# Autodesk Inventor assembly: Finger1
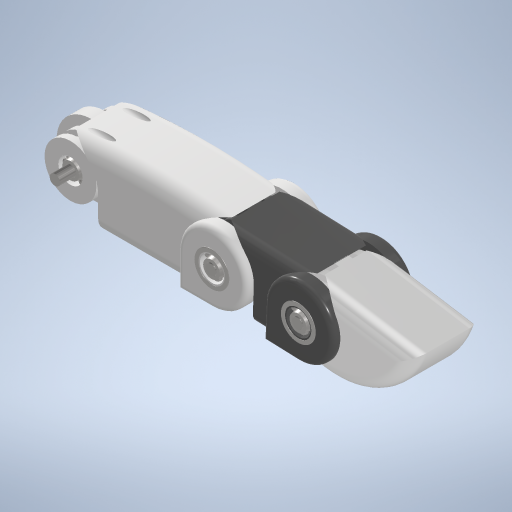
[picture p0: Inventor's stored thumbnail of the model, 512x512]
Saved by Autodesk Inventor 2024 (Build 280153000, 153)
## iProperties
Created: 2024-03-20
Part Number: Finger1
Document SubType Name: Assembly
Designer: Wojtek
Author: Wojtek
## Documents named in this file (6)
- D:\STUDIA\inventor Projects\Bionic_Hand\Fingers\Finger1.iam
- D:\STUDIA\inventor Projects\Bionic_Hand\Fingers\MiddlePart.ipt
- D:\STUDIA\inventor Projects\Bionic_Hand\Fingers\BottomPart.ipt
- C:\Users\Wojtek\OneDrive\Dokumenty\Inventor\Content Center Files\R2024\en-US\Bearing GB_T 292-2007\Rolling bearing B723 AC GB_T 292-2007.ipt
- D:\STUDIA\inventor Projects\Bionic_Hand\Fingers\Roller3mmx25mm.ipt
- D:\STUDIA\inventor Projects\Bionic_Hand\Fingers\TapPart.ipt
## Components (16 placed, 5 different names)
1. MiddlePart:1 — Rigid:1, Rigid:2, Rigid:3, Rigid:4
2. BottomPart:1 — Rigid:5, Rigid:6, Rigid:7, Rigid:8
3. Bearing GB/T 292-2007 Type IN - withdrawn B723 AC:1 — Rigid:1, Rotational:12
4. Bearing GB/T 292-2007 Type IN - withdrawn B723 AC:2 — Rigid:7
5. Bearing GB/T 292-2007 Type IN - withdrawn B723 AC:3 — Rigid:8, Rigid:10
6. Bearing GB/T 292-2007 Type IN - withdrawn B723 AC:4 — Rigid:2
7. Bearing GB/T 292-2007 Type IN - withdrawn B723 AC:5 — Rigid:4
8. Bearing GB/T 292-2007 Type IN - withdrawn B723 AC:6 — Rigid:5, Rigid:9
9. Bearing GB/T 292-2007 Type IN - withdrawn B723 AC:7 — Rigid:6
10. Bearing GB/T 292-2007 Type IN - withdrawn B723 AC:8 — Rigid:3, Rigid:12
11. Roller3mmx25mm:1 — Rigid:9, Rotational:12
12. Roller3mmx25mm:2 — Rigid:10
13. TapPart:1 — Rigid:11, Rotational:13
14. Bearing GB/T 292-2007 Type IN - withdrawn B723 AC:9 — Rigid:11, Rotational:14
15. Bearing GB/T 292-2007 Type IN - withdrawn B723 AC:10 — Rotational:13
16. Roller3mmx25mm:3 — Rigid:12, Rotational:14
## Relationships (15: WeldJoint 12, RevoluteJoint 3)
- Rigid:1 [WeldJoint] (-4 mm): MiddlePart:1 ↔ Bearing GB/T 292-2007 Type IN - withdrawn B723 AC:1
- Rigid:2 [WeldJoint] (-4 mm): MiddlePart:1 ↔ Bearing GB/T 292-2007 Type IN - withdrawn B723 AC:4
- Rigid:3 [WeldJoint]: MiddlePart:1 ↔ Bearing GB/T 292-2007 Type IN - withdrawn B723 AC:8
- Rigid:4 [WeldJoint]: MiddlePart:1 ↔ Bearing GB/T 292-2007 Type IN - withdrawn B723 AC:5
- Rigid:5 [WeldJoint]: BottomPart:1 ↔ Bearing GB/T 292-2007 Type IN - withdrawn B723 AC:6
- Rigid:6 [WeldJoint]: BottomPart:1 ↔ Bearing GB/T 292-2007 Type IN - withdrawn B723 AC:7
- Rigid:7 [WeldJoint] (0.2 mm): BottomPart:1 ↔ Bearing GB/T 292-2007 Type IN - withdrawn B723 AC:2
- Rigid:8 [WeldJoint] (0.2 mm): BottomPart:1 ↔ Bearing GB/T 292-2007 Type IN - withdrawn B723 AC:3
- Rigid:10 [WeldJoint] (20.3 mm): Bearing GB/T 292-2007 Type IN - withdrawn B723 AC:3 ↔ Roller3mmx25mm:2
- Rigid:9 [WeldJoint] (0.25 mm): Bearing GB/T 292-2007 Type IN - withdrawn B723 AC:6 ↔ Roller3mmx25mm:1
- Rotational:12 [RevoluteJoint] (7.7 mm): Bearing GB/T 292-2007 Type IN - withdrawn B723 AC:1 ↔ Roller3mmx25mm:1
- Rigid:11 [WeldJoint] (4 mm): TapPart:1 ↔ Bearing GB/T 292-2007 Type IN - withdrawn B723 AC:9
- Rotational:13 [RevoluteJoint] (4 mm): TapPart:1 ↔ Bearing GB/T 292-2007 Type IN - withdrawn B723 AC:10
- Rigid:12 [WeldJoint] (-0.35 mm): Bearing GB/T 292-2007 Type IN - withdrawn B723 AC:8 ↔ Roller3mmx25mm:3
- Rotational:14 [RevoluteJoint] (7.75 mm): Bearing GB/T 292-2007 Type IN - withdrawn B723 AC:9 ↔ Roller3mmx25mm:3
